# Autodesk Inventor assembly: Assembly_Base_1x1_Magnets
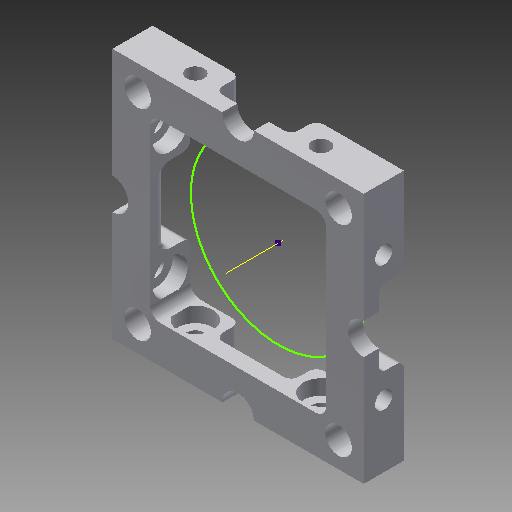
[picture p0: Inventor's stored thumbnail of the model, 512x512]
Saved by Autodesk Inventor 2019 (Build 230136000, 136)
## iProperties
Created: 2019-08-06
Part Number: Assembly_Base_1x1_Magnets
Document SubType Name: Assembly
Designer: marsikovabarbora
Author: marsikovabarbora
## Documents named in this file (3)
- D:\Dropbox\UC2\02_CAD\INVENTOR\uc2_v2\Assembly_Base_1x1_Magnets.iam
- D:\Dropbox\UC2\02_CAD\INVENTOR\uc2_v2\10_Base_v0.ipt
- D:\Dropbox\UC2\02_CAD\INVENTOR\uc2_v2\00_BallMagnets_5mm.ipt
## Components (2 placed, 2 different names)
1. 10_Base_v0:1 — Mate:1
2. 00_BallMagnets_5mm:1 — Mate:1
## Relationships (1: Mate 1)
- Mate:1: 10_Base_v0:1 ↔ 00_BallMagnets_5mm:1
